# Autodesk Inventor assembly: bldc
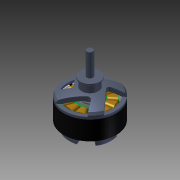
[picture p0: Inventor's stored thumbnail of the model, 180x180]
Saved by Autodesk Inventor 2012 (Build 160160000, 160)
## iProperties
Created: 2014-07-09
Part Number: bldc
Document SubType Name: Assembly
Designer: Anon
Author: Anon
## Documents named in this file (11)
- D:\Dropbox\Courses\GP\git\dronestructure\motor\bldc.iam
- D:\Dropbox\Courses\GP\git\dronestructure\motor\hull.ipt
- D:\Dropbox\Courses\GP\git\dronestructure\motor\magnets.ipt
- D:\Dropbox\Courses\GP\git\dronestructure\motor\cover.ipt
- D:\Dropbox\Courses\GP\git\dronestructure\motor\bearing.ipt
- D:\Dropbox\Courses\GP\git\dronestructure\motor\anchor.ipt
- D:\Dropbox\Courses\GP\git\dronestructure\motor\coils.ipt
- D:\Dropbox\Courses\GP\git\dronestructure\motor\base.ipt
- D:\Dropbox\Courses\GP\git\dronestructure\motor\redlead.ipt
- D:\Dropbox\Courses\GP\git\dronestructure\motor\blacklead.ipt
- D:\Dropbox\Courses\GP\git\dronestructure\motor\bluelead.ipt
## Components (10 placed, 10 different names)
1. hull:1 — Mate:1, Flush:1, Mate:2, Mate:3
2. magnets:1 — Mate:1, Flush:2, Mate:9
3. cover:1 — Mate:2, Mate:3, Mate:6, Mate:9, Flush:9
4. bearing:1 — Mate:4, Flush:6, Flush:8, Flush:10
5. anchor:1 — Mate:4, Mate:5, Flush:4, Mate:8, Flush:6, Mate:12
6. coils:1 — Mate:5, Flush:5, Mate:6, Mate:8, Mate:10
7. base:1 — Mate:10, Flush:7, Flush:11, Flush:12, Angle:1, Mate:15, Mate:16, Mate:19, Mate:23
8. redlead:1 — Mate:17, Mate:18, Angle:4, Mate:20
9. blacklead:1 — Mate:11, Mate:13, Mate:14
10. bluelead:1 — Mate:21, Mate:22, Angle:5, Mate:24
## Relationships (39: Mate 23, Flush 11, Angle 5)
- Mate:1: hull:1 ↔ magnets:1
- Flush:1 (-0.75 mm): hull:1
- Flush:2: magnets:1
- Mate:2: hull:1 ↔ cover:1
- Mate:3: hull:1 ↔ cover:1
- Mate:4: bearing:1 ↔ anchor:1
- Mate:5: anchor:1 ↔ coils:1
- Flush:4 (1.75 mm): anchor:1
- Flush:5: coils:1
- Mate:6: cover:1 ↔ coils:1
- Mate:8: anchor:1 ↔ coils:1
- Mate:9: magnets:1 ↔ cover:1
- Flush:6: bearing:1 ↔ anchor:1
- Mate:10: coils:1 ↔ base:1
- Flush:7 (-0.5 mm): base:1
- Flush:8: bearing:1
- Flush:9 (-8 mm): cover:1
- Flush:10: bearing:1
- Flush:11: base:1
- Flush:12 (-2.5 mm): base:1
- Mate:11: blacklead:1
- Mate:12: anchor:1
- Angle:1 (0 deg): base:1
- Mate:13: blacklead:1
- Mate:14: blacklead:1
- Mate:15: base:1
- Angle:2 (-5 deg)
- Mate:16: base:1
- Angle:3 (-5 deg)
- Mate:17: redlead:1
- Mate:18: redlead:1
- Mate:19: base:1
- Angle:4 (0 deg): redlead:1
- Mate:20: redlead:1
- Mate:21: bluelead:1
- Mate:22: bluelead:1
- Mate:23: base:1
- Angle:5 (0 deg): bluelead:1
- Mate:24: bluelead:1
